# Autodesk Inventor assembly: robot
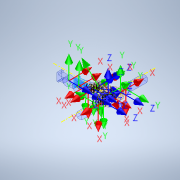
[picture p0: Inventor's stored thumbnail of the model, 180x180]
Saved by Autodesk Inventor 2020.2 (Build 242310000, 310)
## iProperties
Created: 2021-01-29
Part Number: robot
Document SubType Name: Assembly
Designer: DELL
Author: DELL
## Documents named in this file (7)
- D:\repo\FlexipodFast\mesh\v10\robot.iam
- D:\repo\FlexipodFast\mesh\v10\hip.ipt
- D:\repo\FlexipodFast\mesh\v10\thigh.ipt
- D:\repo\FlexipodFast\mesh\v10\shank_back.ipt
- D:\repo\FlexipodFast\mesh\v10\shank_front.ipt
- D:\repo\FlexipodFast\mesh\v10\body.ipt
- D:\repo\FlexipodFast\mesh\v10\knee.ipt
## Components (13 placed, 6 different names)
1. thigh:3 — Rotational:8, Rotational:23
2. thigh:4 — Rotational:12, Angle:36, Rotational:22
3. shank_back:3 — Angle:37, Rotational:24
4. body:1 — Flush:47, Flush:48, Flush:49, Angle:29, Rotational:1, Rotational:2, Rotational:3, Rotational:4, Angle:33, Angle:34, Angle:35, Angle:36, Angle:37
5. knee:1 — Rotational:22, Rotational:24
6. knee:2 — Rotational:23, Rotational:25
7. shank_back:4 — Rotational:25
8. hip:3 — Rotational:3, Rotational:8, Angle:35
9. hip:4 — Angle:29, Rotational:4, Rotational:12
10. hip:1 — Rotational:1, Angle:34, Rotational:26
11. hip:2 — Rotational:2, Angle:33, Rotational:27
12. shank_front:1 — Rotational:26
13. shank_front:2 — Rotational:27
## Relationships (21: RevoluteJoint 12, Angle 6, Flush 3)
- Flush:47: body:1
- Flush:48: body:1
- Flush:49: body:1
- Angle:29 (0 deg): body:1 ↔ hip:4
- Rotational:1 [RevoluteJoint]: body:1 ↔ hip:1
- Rotational:2 [RevoluteJoint]: body:1 ↔ hip:2
- Rotational:3 [RevoluteJoint]: body:1 ↔ hip:3
- Rotational:4 [RevoluteJoint]: body:1 ↔ hip:4
- Rotational:8 [RevoluteJoint]: thigh:3 ↔ hip:3
- Angle:33 (0 deg): body:1 ↔ hip:2
- Angle:34 (180 deg): body:1 ↔ hip:1
- Angle:35 (180 deg): body:1 ↔ hip:3
- Rotational:12 [RevoluteJoint]: thigh:4 ↔ hip:4
- Angle:36 (0 deg): thigh:4 ↔ body:1
- Angle:37 (0 deg): shank_back:3 ↔ body:1
- Rotational:22 [RevoluteJoint]: thigh:4 ↔ knee:1
- Rotational:23 [RevoluteJoint]: thigh:3 ↔ knee:2
- Rotational:24 [RevoluteJoint]: shank_back:3 ↔ knee:1
- Rotational:25 [RevoluteJoint]: knee:2 ↔ shank_back:4
- Rotational:26 [RevoluteJoint]: hip:1 ↔ shank_front:1
- Rotational:27 [RevoluteJoint]: hip:2 ↔ shank_front:2
